# Autodesk Inventor assembly: BigOko
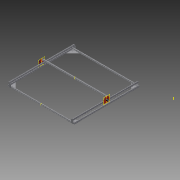
[picture p0: Inventor's stored thumbnail of the model, 180x180]
Saved by Autodesk Inventor 2013 (Build 170138000, 138)
## iProperties
Created: 2013-06-20
Part Number: BigOko
Document SubType Name: Assembly
Designer: Brett
Author: Brett
## Documents named in this file (7)
- C:\Users\Brett\Documents\Autodesk\Projects\Shapeoko_v1i\BigOko.iam
- C:\Users\Brett\Documents\Autodesk\Projects\Shapeoko_v1i\bb_parts\hfs5-2040.ipt
- C:\Users\Brett\Documents\Autodesk\Projects\Shapeoko_v1i\bb_parts\HBLFSSW5-SET.iam
- C:\Users\Brett\Documents\Autodesk\Projects\Shapeoko_v1i\bb_parts\makerslide_1800.ipt
- C:\Users\Brett\Documents\Autodesk\Projects\Shapeoko_v1i\Assemblies\SM-YA01.iam
- C:\Users\Brett\Documents\Autodesk\Projects\Shapeoko_v1i\bb_parts\MAKERSLIDE_RISERS.ipt
- C:\Users\Brett\Documents\Autodesk\Projects\Shapeoko_v1i\bb_parts\GUSSET_200MM.ipt
## Components (21 placed, 6 different names)
1. hfs5-2040:1 — Mate:1, Flush:1, Mate:3, Flush:4, Flush:5, Mate:4, Mate:5, Mate:11, Mate:27, Mate:28, Mate:30
2. hfs5-2040:2 — Mate:2, Flush:2, Flush:3, Flush:6, Mate:7, Mate:9, Mate:15, Mate:22, Mate:24, Mate:31, Mate:33
3. hfs5-2040:3 — Mate:1, Flush:1, Mate:2, Flush:2, Flush:3, Mate:6, Mate:8, Mate:17, Mate:19, Flush:9, Mate:20, Angle:1, Mate:25, Mate:26, Mate:32
4. hfs5-2040:4 — Mate:3, Flush:4, Flush:5, Flush:6, Mate:10, Mate:12, Mate:13, Mate:14, Mate:23, Mate:29
5. HBLFSSW5-SET:1 [sub-assembly] — Mate:4, Mate:5, Mate:6
6. HBLFSSW5-SET:2 [sub-assembly] — Mate:8, Mate:7, Mate:9
7. HBLFSSW5-SET:3 [sub-assembly] — Mate:13, Mate:14, Mate:15
8. HBLFSSW5-SET:4 [sub-assembly] — Mate:10, Mate:11, Mate:12
9. makerslide_1800:1 — Insert:6, Insert:7, Insert:8, Mate:21, Angle:2
10. SM-YA01:1 [sub-assembly] — Tangent:1, Tangent:2, Tangent:3, Insert:6, Insert:7
11. MAKERSLIDE_RISERS:1 — Mate:17, Mate:18, Insert:2
12. MAKERSLIDE_RISERS:2 — Insert:3
13. MAKERSLIDE_RISERS:3 — Mate:19, Flush:9, Insert:4, Insert:5
14. makerslide_1800:2 — Mate:18, Insert:2, Insert:3, Tangent:4, Tangent:5, Tangent:6
15. makerslide_1800:3 — Insert:4, Insert:5, Tangent:1, Tangent:2, Tangent:3, Insert:9, Insert:10
16. SM-YA01:2 [sub-assembly] — Insert:8, Tangent:4, Tangent:5, Tangent:6
17. MAKERSLIDE_RISERS:4 — Insert:9, Insert:10
18. GUSSET_200MM:1 — Mate:22, Mate:23, Mate:24
19. GUSSET_200MM:2 — Mate:25, Mate:26, Mate:27
20. GUSSET_200MM:3 — Mate:31, Mate:32, Mate:33
21. GUSSET_200MM:4 — Mate:28, Mate:29, Mate:30
## Relationships (57: Mate 32, Insert 9, Flush 8, Tangent 6, Angle 2)
- Mate:1: hfs5-2040:1 ↔ hfs5-2040:3
- Flush:1: hfs5-2040:1 ↔ hfs5-2040:3
- Mate:2: hfs5-2040:2 ↔ hfs5-2040:3
- Flush:2: hfs5-2040:2 ↔ hfs5-2040:3
- Flush:3: hfs5-2040:2 ↔ hfs5-2040:3
- Mate:3: hfs5-2040:1 ↔ hfs5-2040:4
- Flush:4: hfs5-2040:1 ↔ hfs5-2040:4
- Flush:5: hfs5-2040:1 ↔ hfs5-2040:4
- Flush:6: hfs5-2040:2 ↔ hfs5-2040:4
- Mate:4: hfs5-2040:1 ↔ HBLFSSW5-SET:1
- Mate:5: hfs5-2040:1 ↔ HBLFSSW5-SET:1
- Mate:6: hfs5-2040:3 ↔ HBLFSSW5-SET:1
- Mate:8: hfs5-2040:3 ↔ HBLFSSW5-SET:2
- Mate:7: hfs5-2040:2 ↔ HBLFSSW5-SET:2
- Mate:9: hfs5-2040:2 ↔ HBLFSSW5-SET:2
- Mate:10: hfs5-2040:4 ↔ HBLFSSW5-SET:4
- Mate:11: hfs5-2040:1 ↔ HBLFSSW5-SET:4
- Mate:12: hfs5-2040:4 ↔ HBLFSSW5-SET:4
- Mate:13: hfs5-2040:4 ↔ HBLFSSW5-SET:3
- Mate:14: hfs5-2040:4 ↔ HBLFSSW5-SET:3
- Mate:15: hfs5-2040:2 ↔ HBLFSSW5-SET:3
- Mate:17: hfs5-2040:3 ↔ MAKERSLIDE_RISERS:1
- Mate:18: MAKERSLIDE_RISERS:1 ↔ makerslide_1800:2
- Insert:2: MAKERSLIDE_RISERS:1 ↔ makerslide_1800:2
- Insert:3: MAKERSLIDE_RISERS:2 ↔ makerslide_1800:2
- Mate:19: hfs5-2040:3 ↔ MAKERSLIDE_RISERS:3
- Flush:9: hfs5-2040:3 ↔ MAKERSLIDE_RISERS:3
- Insert:4: MAKERSLIDE_RISERS:3 ↔ makerslide_1800:3
- Insert:5: MAKERSLIDE_RISERS:3 ↔ makerslide_1800:3
- Tangent:1: SM-YA01:1 ↔ makerslide_1800:3
- Tangent:2: SM-YA01:1 ↔ makerslide_1800:3
- Tangent:3: SM-YA01:1 ↔ makerslide_1800:3
- Insert:6: makerslide_1800:1 ↔ SM-YA01:1
- Insert:7: makerslide_1800:1 ↔ SM-YA01:1
- Insert:8: makerslide_1800:1 ↔ SM-YA01:2
- Tangent:4: makerslide_1800:2 ↔ SM-YA01:2
- Tangent:5: makerslide_1800:2 ↔ SM-YA01:2
- Mate:20: hfs5-2040:3
- Angle:1 (0 deg): hfs5-2040:3
- Mate:21: makerslide_1800:1
- Angle:2 (0 deg): makerslide_1800:1
- Flush:11
- Tangent:6: makerslide_1800:2 ↔ SM-YA01:2
- Insert:9: makerslide_1800:3 ↔ MAKERSLIDE_RISERS:4
- Insert:10: makerslide_1800:3 ↔ MAKERSLIDE_RISERS:4
- Mate:22: hfs5-2040:2 ↔ GUSSET_200MM:1
- Mate:23: hfs5-2040:4 ↔ GUSSET_200MM:1
- Mate:24: hfs5-2040:2 ↔ GUSSET_200MM:1
- Mate:25: hfs5-2040:3 ↔ GUSSET_200MM:2
- Mate:26: hfs5-2040:3 ↔ GUSSET_200MM:2
- Mate:27: hfs5-2040:1 ↔ GUSSET_200MM:2
- Mate:28: hfs5-2040:1 ↔ GUSSET_200MM:4
- Mate:29: hfs5-2040:4 ↔ GUSSET_200MM:4
- Mate:30: hfs5-2040:1 ↔ GUSSET_200MM:4
- Mate:31: hfs5-2040:2 ↔ GUSSET_200MM:3
- Mate:32: hfs5-2040:3 ↔ GUSSET_200MM:3
- Mate:33: hfs5-2040:2 ↔ GUSSET_200MM:3
